# Autodesk Inventor assembly: Assembly1
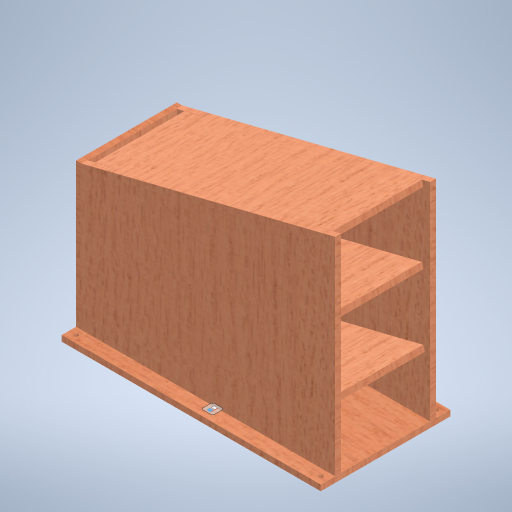
[picture p0: Inventor's stored thumbnail of the model, 512x512]
Saved by Autodesk Inventor 2023 (Build 270158000, 158)
## iProperties
Created: 2023-03-05
Part Number: Assembly1
Document SubType Name: Assembly
Designer: mkhr7
Author: mkhr7
## Documents named in this file (6)
- C:\大学\ロボコンサークル\学ロボ2023\ER_roller_2次ビデオ\Lipo_box\Assembly1.iam
- C:\大学\ロボコンサークル\学ロボ2023\ER_roller_2次ビデオ\Lipo_box\ER_lipo_back_1.ipt
- C:\大学\ロボコンサークル\学ロボ2023\ER_roller_2次ビデオ\Lipo_box\ER_lipo_bottom_1.ipt
- C:\大学\ロボコンサークル\学ロボ2023\ER_roller_2次ビデオ\Lipo_box\ER_lipo_side_2.ipt
- C:\大学\ロボコンサークル\学ロボ2023\ER_roller_2次ビデオ\Lipo_box\ER_lipo_sikiri.ipt
- C:\大学\ロボコンサークル\学ロボ2023\ER_roller_2次ビデオ\Lipo_box\ER_lipo_sikiri_up.ipt
## Components (7 placed, 5 different names)
1. ER_lipo_back_1:1 — メイト:1, メイト:2, フラッシュ:1, フラッシュ:3, フラッシュ:4, フラッシュ:6, メイト:3
2. ER_lipo_bottom_1:1 — メイト:1, メイト:2, フラッシュ:1, フラッシュ:2, フラッシュ:5
3. ER_lipo_side_2:1 — フラッシュ:2, フラッシュ:3, フラッシュ:4, フラッシュ:7, メイト:4, メイト:5, フラッシュ:8, メイト:6, メイト:7, フラッシュ:9, メイト:8, メイト:9
4. ER_lipo_side_2:2 — フラッシュ:5, フラッシュ:6, メイト:3
5. ER_lipo_sikiri:1 — フラッシュ:8, メイト:6, メイト:7
6. ER_lipo_sikiri:2 — フラッシュ:7, メイト:4, メイト:5
7. ER_lipo_sikiri_up:1 — フラッシュ:9, メイト:8, メイト:9
## Relationships (18: Mate 9, Flush 9)
- メイト:1 [Mate]: ER_lipo_back_1:1 ↔ ER_lipo_bottom_1:1
- メイト:2 [Mate]: ER_lipo_back_1:1 ↔ ER_lipo_bottom_1:1
- フラッシュ:1 [Flush]: ER_lipo_back_1:1 ↔ ER_lipo_bottom_1:1
- フラッシュ:2 [Flush]: ER_lipo_bottom_1:1 ↔ ER_lipo_side_2:1
- フラッシュ:3 [Flush]: ER_lipo_back_1:1 ↔ ER_lipo_side_2:1
- フラッシュ:4 [Flush]: ER_lipo_back_1:1 ↔ ER_lipo_side_2:1
- フラッシュ:5 [Flush]: ER_lipo_bottom_1:1 ↔ ER_lipo_side_2:2
- フラッシュ:6 [Flush]: ER_lipo_back_1:1 ↔ ER_lipo_side_2:2
- メイト:3 [Mate]: ER_lipo_back_1:1 ↔ ER_lipo_side_2:2
- フラッシュ:7 [Flush]: ER_lipo_side_2:1 ↔ ER_lipo_sikiri:2
- メイト:4 [Mate]: ER_lipo_side_2:1 ↔ ER_lipo_sikiri:2
- メイト:5 [Mate]: ER_lipo_side_2:1 ↔ ER_lipo_sikiri:2
- フラッシュ:8 [Flush]: ER_lipo_side_2:1 ↔ ER_lipo_sikiri:1
- メイト:6 [Mate]: ER_lipo_side_2:1 ↔ ER_lipo_sikiri:1
- メイト:7 [Mate]: ER_lipo_side_2:1 ↔ ER_lipo_sikiri:1
- フラッシュ:9 [Flush]: ER_lipo_side_2:1 ↔ ER_lipo_sikiri_up:1
- メイト:8 [Mate]: ER_lipo_side_2:1 ↔ ER_lipo_sikiri_up:1
- メイト:9 [Mate]: ER_lipo_side_2:1 ↔ ER_lipo_sikiri_up:1
